# Autodesk Inventor assembly: Arcade
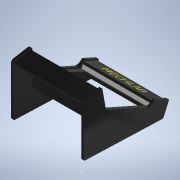
[picture p0: Inventor's stored thumbnail of the model, 180x180]
Saved by Autodesk Inventor 2022 (Build 260153000, 153)
## iProperties
Created: 2023-12-22
Part Number: Arcade
Document SubType Name: Assembly
Designer: Petr Černý
Author: Petr Černý
## Documents named in this file (12)
- C:\Petr\School\VUT Brno\Third_Year\Bachelors_Thesis\git\GamesUI\ArcadeGameMachine\Arcade.iam
- C:\Petr\School\VUT Brno\Third_Year\Bachelors_Thesis\git\GamesUI\ArcadeGameMachine\Monitor.ipt
- C:\Petr\School\VUT Brno\Third_Year\Bachelors_Thesis\git\GamesUI\ArcadeGameMachine\Arcade_Left.ipt
- C:\Petr\School\VUT Brno\Third_Year\Bachelors_Thesis\git\GamesUI\ArcadeGameMachine\Arcade_Right.ipt
- C:\Petr\School\VUT Brno\Third_Year\Bachelors_Thesis\git\GamesUI\ArcadeGameMachine\Arcade_Front.ipt
- C:\Petr\School\VUT Brno\Third_Year\Bachelors_Thesis\git\GamesUI\ArcadeGameMachine\Arcade_ControlTop.ipt
- C:\Petr\School\VUT Brno\Third_Year\Bachelors_Thesis\git\GamesUI\ArcadeGameMachine\Arcade_MonitorStand.ipt
- C:\Petr\School\VUT Brno\Third_Year\Bachelors_Thesis\git\GamesUI\ArcadeGameMachine\Arcade_TopName.ipt
- C:\Petr\School\VUT Brno\Third_Year\Bachelors_Thesis\git\GamesUI\ArcadeGameMachine\Arcade_FrontBottom.ipt
- C:\Petr\School\VUT Brno\Third_Year\Bachelors_Thesis\git\GamesUI\ArcadeGameMachine\Arcade_TopFill.ipt
- C:\Petr\School\VUT Brno\Third_Year\Bachelors_Thesis\git\GamesUI\ArcadeGameMachine\Arcade_top.ipt
- C:\Petr\School\VUT Brno\Third_Year\Bachelors_Thesis\git\GamesUI\ArcadeGameMachine\Arcade_MonitorMount.ipt
## Components (11 placed, 11 different names)
1. Monitor:1 — Flush:1, Flush:2, Mate:28
2. Arcade_Left:1 — Mate:1, Mate:2, Mate:3, Flush:4, Flush:5, Mate:9, Mate:10, Mate:12, Mate:13, Mate:14, Mate:16, Mate:17, Mate:18, Mate:20, Mate:21, Mate:22, Mate:23
3. Arcade_Right:1 — Flush:4, Flush:5, Mate:5, Mate:6, Mate:7, Mate:8, Mate:15, Mate:25, Mate:26, Mate:29
4. Arcade_Front:1 — Mate:1, Mate:2, Mate:3, Flush:1, Flush:2, Mate:5, Mate:19, Mate:27, Mate:28
5. Arcade_ControlTop:1 — Mate:6, Mate:7, Mate:8
6. Arcade_MonitorStand:1 — Mate:9, Mate:10, Mate:27
7. Arcade_TopName:1 — Mate:12, Mate:13, Mate:14
8. Arcade_FrontBottom:1 — Mate:15, Mate:16, Mate:17
9. Arcade_TopFill:1 — Mate:18, Mate:19, Mate:20
10. Arcade_Top:1 — Mate:21, Mate:22, Mate:23
11. Arcade_MonitorMount:1 — Mate:25, Mate:26, Mate:29
## Relationships (30: Mate 26, Flush 4)
- Mate:1: Arcade_Left:1 ↔ Arcade_Front:1
- Mate:2: Arcade_Left:1 ↔ Arcade_Front:1
- Mate:3: Arcade_Left:1 ↔ Arcade_Front:1
- Flush:1: Monitor:1 ↔ Arcade_Front:1
- Flush:2: Monitor:1 ↔ Arcade_Front:1
- Flush:4: Arcade_Left:1 ↔ Arcade_Right:1
- Flush:5: Arcade_Left:1 ↔ Arcade_Right:1
- Mate:5: Arcade_Right:1 ↔ Arcade_Front:1
- Mate:6: Arcade_Right:1 ↔ Arcade_ControlTop:1
- Mate:7: Arcade_Right:1 ↔ Arcade_ControlTop:1
- Mate:8: Arcade_Right:1 ↔ Arcade_ControlTop:1
- Mate:9: Arcade_Left:1 ↔ Arcade_MonitorStand:1
- Mate:10: Arcade_Left:1 ↔ Arcade_MonitorStand:1
- Mate:12: Arcade_Left:1 ↔ Arcade_TopName:1
- Mate:13: Arcade_Left:1 ↔ Arcade_TopName:1
- Mate:14: Arcade_Left:1 ↔ Arcade_TopName:1
- Mate:15: Arcade_Right:1 ↔ Arcade_FrontBottom:1
- Mate:16: Arcade_Left:1 ↔ Arcade_FrontBottom:1
- Mate:17: Arcade_Left:1 ↔ Arcade_FrontBottom:1
- Mate:18: Arcade_Left:1 ↔ Arcade_TopFill:1
- Mate:19: Arcade_Front:1 ↔ Arcade_TopFill:1
- Mate:20: Arcade_Left:1 ↔ Arcade_TopFill:1
- Mate:21: Arcade_Left:1 ↔ Arcade_Top:1
- Mate:22: Arcade_Left:1 ↔ Arcade_Top:1
- Mate:23: Arcade_Left:1 ↔ Arcade_Top:1
- Mate:25: Arcade_Right:1 ↔ Arcade_MonitorMount:1
- Mate:26: Arcade_Right:1 ↔ Arcade_MonitorMount:1
- Mate:27: Arcade_Front:1 ↔ Arcade_MonitorStand:1
- Mate:28: Monitor:1 ↔ Arcade_Front:1
- Mate:29: Arcade_Right:1 ↔ Arcade_MonitorMount:1
